# Autodesk Inventor assembly: Slidey Mecanum L thing V2
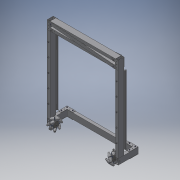
[picture p0: Inventor's stored thumbnail of the model, 180x180]
Saved by Autodesk Inventor 2018 (Build 220112000, 112)
## iProperties
Created: 2019-01-11
Part Number: Slidey Mecanum L thing V2
Document SubType Name: Assembly
Designer: s-2512711
Author: s-2512711
## Documents named in this file (12)
- C:\Users\maste\OneDrive\Documents\GitHub\2019CAD\Drivebase but Calvin is a mad man\Slidey Mecanum L thing V2.iam
- C:\Users\maste\OneDrive\Documents\GitHub\2019CAD\Drivebase but Calvin is a mad man\1X2 7in.ipt
- C:\Users\maste\OneDrive\Documents\GitHub\2019CAD\Drivebase but Calvin is a mad man\1x2 28in.ipt
- C:\Users\maste\OneDrive\Documents\GitHub\2019CAD\Drivebase but Calvin is a mad man\1x2 30in.ipt
- C:\Users\maste\OneDrive\Documents\GitHub\2019CAD\Drivebase but Calvin is a mad man\4_Mecanum_Wheel_Left_217-3644.iam
- C:\Users\maste\OneDrive\Documents\GitHub\2019CAD\Drivebase but Calvin is a mad man\4_Mecanum_Wheel_Right_217-3645.iam
- C:\Users\maste\OneDrive\Documents\GitHub\2019CAD\Drivebase but Calvin is a mad man\Strutural Integrity Bar.ipt
- C:\Users\maste\OneDrive\Documents\GitHub\2019CAD\Drivebase but Calvin is a mad man\WS_10_40_610_4.ipt
- C:\Users\maste\OneDrive\Documents\GitHub\2019CAD\Drivebase but Calvin is a mad man\91831A011_TYPE 18-8 STAINLESS STL NYLON-INSERT LOCKNUT.ipt
- C:\Users\maste\OneDrive\Documents\GitHub\2019CAD\Drivebase but Calvin is a mad man\73434-Fastenal-01-12-2019.ipt
- C:\Users\maste\OneDrive\Documents\GitHub\2019CAD\Drivebase but Calvin is a mad man\L gusset.ipt
- C:\Users\maste\OneDrive\Documents\GitHub\2019CAD\Drivebase but Calvin is a mad man\C-Bracket.ipt
## Components (61 placed, 11 different names)
1. 1X2 7in:1 — Mate:4, Mate:5, Mate:6, Mate:7, Mate:8, Mate:9, Mate:22, Mate:23, Mate:24, Mate:55, Mate:57, Mate:58, Mate:60
2. 1X2 7in:2 — Mate:1, Mate:2, Mate:3, Mate:10, Mate:11, Mate:12, Mate:25, Mate:26, Mate:27, Mate:49, Mate:50, Mate:52, Mate:54
3. 1x2 28in:1 — Mate:7, Mate:8, Mate:9, Mate:10, Mate:11, Mate:12, Mate:51, Mate:53, Mate:56, Mate:59
4. 1x2 28in:2 — Mate:16, Mate:17, Flush:1, Mate:29, Mate:31, Mate:127, Mate:130, Mate:133, Mate:136, Angle:1, Angle:2
5. 1x2 28in:3 — Mate:13, Mate:14, Mate:15, Flush:1, Mate:126, Mate:129
6. 1x2 30in:1 — Mate:4, Mate:5, Mate:6, Mate:28, Flush:2, Mate:115, Mate:116, Mate:117, Mate:118, Mate:119, Mate:131, Mate:132, Mate:134, Mate:135
7. 1x2 30in:2 — Mate:1, Mate:2, Mate:3, Mate:13, Mate:14, Mate:15, Mate:16, Mate:17, Mate:30, Flush:3, Mate:120, Mate:121, Mate:122, Mate:123, Mate:124, Mate:125, Mate:128
8. 4_Mecanum_Wheel_Left_217-3644:1 [sub-assembly] — Mate:22, Mate:23, Mate:24
9. 4_Mecanum_Wheel_Right_217-3645:1 [sub-assembly] — Mate:25, Mate:26, Mate:27
10. Strutural Integrity Bar:1 — Mate:137, Mate:138, Angle:1, Mate:141, Mate:142, Mate:147, Mate:148
11. Strutural Integrity Bar:2 — Mate:139, Mate:140, Angle:2, Mate:143, Mate:144, Mate:145, Mate:146
12. WS_10_40_610_4:1 — Mate:30, Mate:31, Flush:3, Mate:90, Mate:91, Mate:92, Mate:93, Mate:94, Mate:95, Mate:96, Mate:97, Mate:98, Mate:99
13. WS_10_40_610_4:2 — Mate:28, Mate:29, Flush:2, Mate:85, Mate:86, Mate:87, Mate:88, Mate:89, Mate:100, Mate:101, Mate:102, Mate:103, Mate:104
14. 91831A011_TYPE 18-8 STAINLESS STL NYLON-INSERT LOCKNUT:1 — Mate:150, Mate:156
15. 91831A011_TYPE 18-8 STAINLESS STL NYLON-INSERT LOCKNUT:2 — Mate:152, Mate:153
16. 73434-Fastenal-01-12-2019:1 — Mate:144, Mate:145, Mate:153
17. 73434-Fastenal-01-12-2019:2 — Mate:143, Mate:146, Mate:156
18. 73434-Fastenal-01-12-2019:3 — Mate:141, Mate:147, Mate:155
19. 73434-Fastenal-01-12-2019:4 — Mate:142, Mate:148, Mate:154
20. 91831A011_TYPE 18-8 STAINLESS STL NYLON-INSERT LOCKNUT:3 — Mate:151, Mate:154
21. 91831A011_TYPE 18-8 STAINLESS STL NYLON-INSERT LOCKNUT:4 — Mate:149, Mate:155
22. 91831A011_TYPE 18-8 STAINLESS STL NYLON-INSERT LOCKNUT:5 — Mate:68, Mate:71
23. 91831A011_TYPE 18-8 STAINLESS STL NYLON-INSERT LOCKNUT:6 — Mate:69, Mate:72
24. 91831A011_TYPE 18-8 STAINLESS STL NYLON-INSERT LOCKNUT:7 — Mate:67, Mate:70
25. 91831A011_TYPE 18-8 STAINLESS STL NYLON-INSERT LOCKNUT:8 — Mate:81, Mate:82
26. 91831A011_TYPE 18-8 STAINLESS STL NYLON-INSERT LOCKNUT:9 — Mate:80, Mate:83
27. 91831A011_TYPE 18-8 STAINLESS STL NYLON-INSERT LOCKNUT:10 — Mate:79, Mate:84
28. 73434-Fastenal-01-12-2019:5 — Mate:74, Mate:77, Mate:80
29. 73434-Fastenal-01-12-2019:6 — Mate:73, Mate:78, Mate:79
30. 73434-Fastenal-01-12-2019:7 — Mate:75, Mate:76, Mate:81
31. 73434-Fastenal-01-12-2019:8 — Mate:65, Mate:66, Mate:69
32. 73434-Fastenal-01-12-2019:9 — Mate:63, Mate:64, Mate:68
33. 73434-Fastenal-01-12-2019:10 — Mate:61, Mate:62, Mate:67
34. L gusset:1 — Mate:49, Mate:50, Mate:51, Mate:73, Mate:74, Mate:75, Mate:76, Mate:77, Mate:78
35. L gusset:2 — Mate:52, Mate:53, Mate:54, Mate:82, Mate:83, Mate:84
36. L gusset:3 — Mate:58, Mate:59, Mate:60, Mate:70, Mate:71, Mate:72
37. L gusset:4 — Mate:55, Mate:56, Mate:57, Mate:61, Mate:62, Mate:63, Mate:64, Mate:65, Mate:66
38. 91831A011_TYPE 18-8 STAINLESS STL NYLON-INSERT LOCKNUT:11 — Mate:111, Mate:121
39. 91831A011_TYPE 18-8 STAINLESS STL NYLON-INSERT LOCKNUT:12 — Mate:110, Mate:120
40. 91831A011_TYPE 18-8 STAINLESS STL NYLON-INSERT LOCKNUT:13 — Mate:105, Mate:115
41. 91831A011_TYPE 18-8 STAINLESS STL NYLON-INSERT LOCKNUT:14 — Mate:106, Mate:116
42. 91831A011_TYPE 18-8 STAINLESS STL NYLON-INSERT LOCKNUT:15 — Mate:107, Mate:117
43. 91831A011_TYPE 18-8 STAINLESS STL NYLON-INSERT LOCKNUT:16 — Mate:108, Mate:118
44. 91831A011_TYPE 18-8 STAINLESS STL NYLON-INSERT LOCKNUT:17 — Mate:109, Mate:119
45. 91831A011_TYPE 18-8 STAINLESS STL NYLON-INSERT LOCKNUT:18 — Mate:114, Mate:124
46. 91831A011_TYPE 18-8 STAINLESS STL NYLON-INSERT LOCKNUT:19 — Mate:113, Mate:123
47. 91831A011_TYPE 18-8 STAINLESS STL NYLON-INSERT LOCKNUT:20 — Mate:112, Mate:122
48. 73434-Fastenal-01-12-2019:11 — Mate:85, Mate:104, Mate:105
49. 73434-Fastenal-01-12-2019:12 — Mate:86, Mate:103, Mate:106
50. 73434-Fastenal-01-12-2019:13 — Mate:87, Mate:102, Mate:107
51. 73434-Fastenal-01-12-2019:14 — Mate:89, Mate:100, Mate:109
52. 73434-Fastenal-01-12-2019:15 — Mate:88, Mate:101, Mate:108
53. 73434-Fastenal-01-12-2019:16 — Mate:94, Mate:95, Mate:114
54. 73434-Fastenal-01-12-2019:17 — Mate:93, Mate:96, Mate:113
55. 73434-Fastenal-01-12-2019:18 — Mate:92, Mate:97, Mate:112
56. 73434-Fastenal-01-12-2019:19 — Mate:91, Mate:98, Mate:111
57. 73434-Fastenal-01-12-2019:20 — Mate:90, Mate:99, Mate:110
58. C-Bracket:1 — Mate:131, Mate:132, Mate:133, Mate:137, Mate:138, Mate:150
59. C-Bracket:2 — Mate:134, Mate:135, Mate:136, Mate:149
60. C-Bracket:3 — Mate:128, Mate:129, Mate:130, Mate:139, Mate:140, Mate:151
61. C-Bracket:4 — Mate:125, Mate:126, Mate:127, Mate:152
## Relationships (140: Mate 135, Flush 3, Angle 2)
- Mate:1: 1X2 7in:2 ↔ 1x2 30in:2
- Mate:2: 1X2 7in:2 ↔ 1x2 30in:2
- Mate:3: 1X2 7in:2 ↔ 1x2 30in:2
- Mate:4: 1X2 7in:1 ↔ 1x2 30in:1
- Mate:5: 1X2 7in:1 ↔ 1x2 30in:1
- Mate:6: 1X2 7in:1 ↔ 1x2 30in:1
- Mate:7: 1X2 7in:1 ↔ 1x2 28in:1
- Mate:8: 1X2 7in:1 ↔ 1x2 28in:1
- Mate:9: 1X2 7in:1 ↔ 1x2 28in:1
- Mate:10: 1X2 7in:2 ↔ 1x2 28in:1
- Mate:11: 1X2 7in:2 ↔ 1x2 28in:1
- Mate:12: 1X2 7in:2 ↔ 1x2 28in:1
- Mate:13: 1x2 28in:3 ↔ 1x2 30in:2
- Mate:14: 1x2 28in:3 ↔ 1x2 30in:2
- Mate:15: 1x2 28in:3 ↔ 1x2 30in:2
- Mate:16: 1x2 28in:2 ↔ 1x2 30in:2
- Mate:17: 1x2 28in:2 ↔ 1x2 30in:2
- Flush:1 (50.8 mm): 1x2 28in:2 ↔ 1x2 28in:3
- Mate:22: 1X2 7in:1 ↔ 4_Mecanum_Wheel_Left_217-3644:1
- Mate:23: 1X2 7in:1 ↔ 4_Mecanum_Wheel_Left_217-3644:1
- Mate:24: 1X2 7in:1 ↔ 4_Mecanum_Wheel_Left_217-3644:1
- Mate:25: 1X2 7in:2 ↔ 4_Mecanum_Wheel_Right_217-3645:1
- Mate:26: 1X2 7in:2 ↔ 4_Mecanum_Wheel_Right_217-3645:1
- Mate:27: 1X2 7in:2 ↔ 4_Mecanum_Wheel_Right_217-3645:1
- Mate:28: 1x2 30in:1 ↔ WS_10_40_610_4:2
- Mate:29 (25.4 mm): 1x2 28in:2 ↔ WS_10_40_610_4:2
- Flush:2 (-7.3025 mm): 1x2 30in:1 ↔ WS_10_40_610_4:2
- Mate:30: 1x2 30in:2 ↔ WS_10_40_610_4:1
- Mate:31 (25.4 mm): 1x2 28in:2 ↔ WS_10_40_610_4:1
- Flush:3 (-7.3025 mm): 1x2 30in:2 ↔ WS_10_40_610_4:1
- Mate:49: 1X2 7in:2 ↔ L gusset:1
- Mate:50: 1X2 7in:2 ↔ L gusset:1
- Mate:51: 1x2 28in:1 ↔ L gusset:1
- Mate:52: 1X2 7in:2 ↔ L gusset:2
- Mate:53: 1x2 28in:1 ↔ L gusset:2
- Mate:54: 1X2 7in:2 ↔ L gusset:2
- Mate:55: 1X2 7in:1 ↔ L gusset:4
- Mate:56: 1x2 28in:1 ↔ L gusset:4
- Mate:57: 1X2 7in:1 ↔ L gusset:4
- Mate:58: 1X2 7in:1 ↔ L gusset:3
- Mate:59: 1x2 28in:1 ↔ L gusset:3
- Mate:60: 1X2 7in:1 ↔ L gusset:3
- Mate:61: 73434-Fastenal-01-12-2019:10 ↔ L gusset:4
- Mate:62: 73434-Fastenal-01-12-2019:10 ↔ L gusset:4
- Mate:63: 73434-Fastenal-01-12-2019:9 ↔ L gusset:4
- Mate:64: 73434-Fastenal-01-12-2019:9 ↔ L gusset:4
- Mate:65: 73434-Fastenal-01-12-2019:8 ↔ L gusset:4
- Mate:66: 73434-Fastenal-01-12-2019:8 ↔ L gusset:4
- Mate:67: 91831A011_TYPE 18-8 STAINLESS STL NYLON-INSERT LOCKNUT:7 ↔ 73434-Fastenal-01-12-2019:10
- Mate:68: 91831A011_TYPE 18-8 STAINLESS STL NYLON-INSERT LOCKNUT:5 ↔ 73434-Fastenal-01-12-2019:9
- Mate:69: 91831A011_TYPE 18-8 STAINLESS STL NYLON-INSERT LOCKNUT:6 ↔ 73434-Fastenal-01-12-2019:8
- Mate:70: 91831A011_TYPE 18-8 STAINLESS STL NYLON-INSERT LOCKNUT:7 ↔ L gusset:3
- Mate:71: 91831A011_TYPE 18-8 STAINLESS STL NYLON-INSERT LOCKNUT:5 ↔ L gusset:3
- Mate:72: 91831A011_TYPE 18-8 STAINLESS STL NYLON-INSERT LOCKNUT:6 ↔ L gusset:3
- Mate:73: 73434-Fastenal-01-12-2019:6 ↔ L gusset:1
- Mate:74: 73434-Fastenal-01-12-2019:5 ↔ L gusset:1
- Mate:75: 73434-Fastenal-01-12-2019:7 ↔ L gusset:1
- Mate:76: 73434-Fastenal-01-12-2019:7 ↔ L gusset:1
- Mate:77: 73434-Fastenal-01-12-2019:5 ↔ L gusset:1
- Mate:78: 73434-Fastenal-01-12-2019:6 ↔ L gusset:1
- Mate:79: 91831A011_TYPE 18-8 STAINLESS STL NYLON-INSERT LOCKNUT:10 ↔ 73434-Fastenal-01-12-2019:6
- Mate:80: 91831A011_TYPE 18-8 STAINLESS STL NYLON-INSERT LOCKNUT:9 ↔ 73434-Fastenal-01-12-2019:5
- Mate:81: 91831A011_TYPE 18-8 STAINLESS STL NYLON-INSERT LOCKNUT:8 ↔ 73434-Fastenal-01-12-2019:7
- Mate:82: 91831A011_TYPE 18-8 STAINLESS STL NYLON-INSERT LOCKNUT:8 ↔ L gusset:2
- Mate:83: 91831A011_TYPE 18-8 STAINLESS STL NYLON-INSERT LOCKNUT:9 ↔ L gusset:2
- Mate:84: 91831A011_TYPE 18-8 STAINLESS STL NYLON-INSERT LOCKNUT:10 ↔ L gusset:2
- Mate:85: WS_10_40_610_4:2 ↔ 73434-Fastenal-01-12-2019:11
- Mate:86: WS_10_40_610_4:2 ↔ 73434-Fastenal-01-12-2019:12
- Mate:87: WS_10_40_610_4:2 ↔ 73434-Fastenal-01-12-2019:13
- Mate:88: WS_10_40_610_4:2 ↔ 73434-Fastenal-01-12-2019:15
- Mate:89: WS_10_40_610_4:2 ↔ 73434-Fastenal-01-12-2019:14
- Mate:90: WS_10_40_610_4:1 ↔ 73434-Fastenal-01-12-2019:20
- Mate:91: WS_10_40_610_4:1 ↔ 73434-Fastenal-01-12-2019:19
- Mate:92: WS_10_40_610_4:1 ↔ 73434-Fastenal-01-12-2019:18
- Mate:93: WS_10_40_610_4:1 ↔ 73434-Fastenal-01-12-2019:17
- Mate:94: WS_10_40_610_4:1 ↔ 73434-Fastenal-01-12-2019:16
- Mate:95: WS_10_40_610_4:1 ↔ 73434-Fastenal-01-12-2019:16
- Mate:96: WS_10_40_610_4:1 ↔ 73434-Fastenal-01-12-2019:17
- Mate:97: WS_10_40_610_4:1 ↔ 73434-Fastenal-01-12-2019:18
- Mate:98: WS_10_40_610_4:1 ↔ 73434-Fastenal-01-12-2019:19
- Mate:99: WS_10_40_610_4:1 ↔ 73434-Fastenal-01-12-2019:20
- Mate:100: WS_10_40_610_4:2 ↔ 73434-Fastenal-01-12-2019:14
- Mate:101: WS_10_40_610_4:2 ↔ 73434-Fastenal-01-12-2019:15
- Mate:102: WS_10_40_610_4:2 ↔ 73434-Fastenal-01-12-2019:13
- Mate:103: WS_10_40_610_4:2 ↔ 73434-Fastenal-01-12-2019:12
- Mate:104: WS_10_40_610_4:2 ↔ 73434-Fastenal-01-12-2019:11
- Mate:105: 91831A011_TYPE 18-8 STAINLESS STL NYLON-INSERT LOCKNUT:13 ↔ 73434-Fastenal-01-12-2019:11
- Mate:106: 91831A011_TYPE 18-8 STAINLESS STL NYLON-INSERT LOCKNUT:14 ↔ 73434-Fastenal-01-12-2019:12
- Mate:107: 91831A011_TYPE 18-8 STAINLESS STL NYLON-INSERT LOCKNUT:15 ↔ 73434-Fastenal-01-12-2019:13
- Mate:108: 91831A011_TYPE 18-8 STAINLESS STL NYLON-INSERT LOCKNUT:16 ↔ 73434-Fastenal-01-12-2019:15
- Mate:109: 91831A011_TYPE 18-8 STAINLESS STL NYLON-INSERT LOCKNUT:17 ↔ 73434-Fastenal-01-12-2019:14
- Mate:110: 91831A011_TYPE 18-8 STAINLESS STL NYLON-INSERT LOCKNUT:12 ↔ 73434-Fastenal-01-12-2019:20
- Mate:111: 91831A011_TYPE 18-8 STAINLESS STL NYLON-INSERT LOCKNUT:11 ↔ 73434-Fastenal-01-12-2019:19
- Mate:112: 91831A011_TYPE 18-8 STAINLESS STL NYLON-INSERT LOCKNUT:20 ↔ 73434-Fastenal-01-12-2019:18
- Mate:113: 91831A011_TYPE 18-8 STAINLESS STL NYLON-INSERT LOCKNUT:19 ↔ 73434-Fastenal-01-12-2019:17
- Mate:114: 91831A011_TYPE 18-8 STAINLESS STL NYLON-INSERT LOCKNUT:18 ↔ 73434-Fastenal-01-12-2019:16
- Mate:115: 1x2 30in:1 ↔ 91831A011_TYPE 18-8 STAINLESS STL NYLON-INSERT LOCKNUT:13
- Mate:116: 1x2 30in:1 ↔ 91831A011_TYPE 18-8 STAINLESS STL NYLON-INSERT LOCKNUT:14
- Mate:117: 1x2 30in:1 ↔ 91831A011_TYPE 18-8 STAINLESS STL NYLON-INSERT LOCKNUT:15
- Mate:118: 1x2 30in:1 ↔ 91831A011_TYPE 18-8 STAINLESS STL NYLON-INSERT LOCKNUT:16
- Mate:119: 1x2 30in:1 ↔ 91831A011_TYPE 18-8 STAINLESS STL NYLON-INSERT LOCKNUT:17
- Mate:120: 1x2 30in:2 ↔ 91831A011_TYPE 18-8 STAINLESS STL NYLON-INSERT LOCKNUT:12
- Mate:121: 1x2 30in:2 ↔ 91831A011_TYPE 18-8 STAINLESS STL NYLON-INSERT LOCKNUT:11
- Mate:122: 1x2 30in:2 ↔ 91831A011_TYPE 18-8 STAINLESS STL NYLON-INSERT LOCKNUT:20
- Mate:123: 1x2 30in:2 ↔ 91831A011_TYPE 18-8 STAINLESS STL NYLON-INSERT LOCKNUT:19
- Mate:124: 1x2 30in:2 ↔ 91831A011_TYPE 18-8 STAINLESS STL NYLON-INSERT LOCKNUT:18
- Mate:125: 1x2 30in:2 ↔ C-Bracket:4
- Mate:126: 1x2 28in:3 ↔ C-Bracket:4
- Mate:127: 1x2 28in:2 ↔ C-Bracket:4
- Mate:128: 1x2 30in:2 ↔ C-Bracket:3
- Mate:129: 1x2 28in:3 ↔ C-Bracket:3
- Mate:130: 1x2 28in:2 ↔ C-Bracket:3
- Mate:131: 1x2 30in:1 ↔ C-Bracket:1
- Mate:132: 1x2 30in:1 ↔ C-Bracket:1
- Mate:133: 1x2 28in:2 ↔ C-Bracket:1
- Mate:134: 1x2 30in:1 ↔ C-Bracket:2
- Mate:135: 1x2 30in:1 ↔ C-Bracket:2
- Mate:136: 1x2 28in:2 ↔ C-Bracket:2
- Mate:137: Strutural Integrity Bar:1 ↔ C-Bracket:1
- Mate:138: Strutural Integrity Bar:1 ↔ C-Bracket:1
- Angle:1 (-5.19 deg): 1x2 28in:2 ↔ Strutural Integrity Bar:1
- Mate:139: Strutural Integrity Bar:2 ↔ C-Bracket:3
- Mate:140: Strutural Integrity Bar:2 ↔ C-Bracket:3
- Angle:2 (-5.19 deg): 1x2 28in:2 ↔ Strutural Integrity Bar:2
- Mate:141: Strutural Integrity Bar:1 ↔ 73434-Fastenal-01-12-2019:3
- Mate:142: Strutural Integrity Bar:1 ↔ 73434-Fastenal-01-12-2019:4
- Mate:143: Strutural Integrity Bar:2 ↔ 73434-Fastenal-01-12-2019:2
- Mate:144: Strutural Integrity Bar:2 ↔ 73434-Fastenal-01-12-2019:1
- Mate:145: Strutural Integrity Bar:2 ↔ 73434-Fastenal-01-12-2019:1
- Mate:146: Strutural Integrity Bar:2 ↔ 73434-Fastenal-01-12-2019:2
- Mate:147: Strutural Integrity Bar:1 ↔ 73434-Fastenal-01-12-2019:3
- Mate:148: Strutural Integrity Bar:1 ↔ 73434-Fastenal-01-12-2019:4
- Mate:149: 91831A011_TYPE 18-8 STAINLESS STL NYLON-INSERT LOCKNUT:4 ↔ C-Bracket:2
- Mate:150: 91831A011_TYPE 18-8 STAINLESS STL NYLON-INSERT LOCKNUT:1 ↔ C-Bracket:1
- Mate:151: 91831A011_TYPE 18-8 STAINLESS STL NYLON-INSERT LOCKNUT:3 ↔ C-Bracket:3
- Mate:152: 91831A011_TYPE 18-8 STAINLESS STL NYLON-INSERT LOCKNUT:2 ↔ C-Bracket:4
- Mate:153: 91831A011_TYPE 18-8 STAINLESS STL NYLON-INSERT LOCKNUT:2 ↔ 73434-Fastenal-01-12-2019:1
- Mate:154: 73434-Fastenal-01-12-2019:4 ↔ 91831A011_TYPE 18-8 STAINLESS STL NYLON-INSERT LOCKNUT:3
- Mate:155: 73434-Fastenal-01-12-2019:3 ↔ 91831A011_TYPE 18-8 STAINLESS STL NYLON-INSERT LOCKNUT:4
- Mate:156: 91831A011_TYPE 18-8 STAINLESS STL NYLON-INSERT LOCKNUT:1 ↔ 73434-Fastenal-01-12-2019:2
